# Autodesk Inventor assembly: spielfeld_gesamt
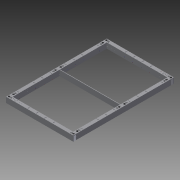
[picture p0: Inventor's stored thumbnail of the model, 180x180]
Saved by Autodesk Inventor 2015 (Build 190159000, 159)
## iProperties
Created: 2018-04-09
Part Number: spielfeld_gesamt
Document SubType Name: Assembly
Designer: wepet
Author: wepet
## Documents named in this file (5)
- C:\workspace\robosax\licht\Alles\spielfeld_gesamt.iam
- C:\workspace\robosax\licht\Einzelteil_150\licht_150.iam
- C:\workspace\robosax\licht\Einzelteil_200\licht_200.iam
- C:\workspace\robosax\licht\Alles\licht_150_MIR.iam
- C:\workspace\robosax\licht\Alles\spielfeld_trennwand.ipt
## Components (7 placed, 4 different names)
1. licht_150:1 [sub-assembly] — Passend:1, Fluchtend:1, Fluchtend:2, Fluchtend:3, Fluchtend:4
2. licht_150:2 [sub-assembly] — Passend:3, Fluchtend:7, Fluchtend:8, Fluchtend:9, Fluchtend:10, Fluchtend:11, Fluchtend:12, Passend:5
3. licht_200:1 [sub-assembly] — Passend:1, Fluchtend:1, Fluchtend:2, Passend:4
4. licht_200:2 [sub-assembly] — Passend:2, Fluchtend:5, Fluchtend:6, Passend:3, Fluchtend:7, Fluchtend:8
5. licht_150_MIR:1 [sub-assembly] — Fluchtend:3, Fluchtend:4, Passend:2, Fluchtend:5, Fluchtend:6
6. licht_150_MIR:2 [sub-assembly] — Fluchtend:9, Fluchtend:10, Passend:4, Passend:6
7. spielfeld_trennwand:1 — Fluchtend:11, Fluchtend:12, Passend:5, Passend:6
## Relationships (18: Flush 12, Mate 6)
- Passend:1 [Mate]: licht_150:1 ↔ licht_200:1
- Fluchtend:1 [Flush]: licht_150:1 ↔ licht_200:1
- Fluchtend:2 [Flush]: licht_150:1 ↔ licht_200:1
- Fluchtend:3 [Flush]: licht_150:1 ↔ licht_150_MIR:1
- Fluchtend:4 [Flush]: licht_150:1 ↔ licht_150_MIR:1
- Passend:2 [Mate]: licht_200:2 ↔ licht_150_MIR:1
- Fluchtend:5 [Flush]: licht_200:2 ↔ licht_150_MIR:1
- Fluchtend:6 [Flush]: licht_200:2 ↔ licht_150_MIR:1
- Passend:3 [Mate]: licht_150:2 ↔ licht_200:2
- Fluchtend:7 [Flush]: licht_150:2 ↔ licht_200:2
- Fluchtend:8 [Flush]: licht_150:2 ↔ licht_200:2
- Fluchtend:9 [Flush]: licht_150:2 ↔ licht_150_MIR:2
- Fluchtend:10 [Flush]: licht_150:2 ↔ licht_150_MIR:2
- Passend:4 [Mate]: licht_200:1 ↔ licht_150_MIR:2
- Fluchtend:11 [Flush]: licht_150:2 ↔ spielfeld_trennwand:1
- Fluchtend:12 [Flush]: licht_150:2 ↔ spielfeld_trennwand:1
- Passend:5 [Mate]: licht_150:2 ↔ spielfeld_trennwand:1
- Passend:6 [Mate]: licht_150_MIR:2 ↔ spielfeld_trennwand:1
